# Autodesk Inventor assembly: EX_ONE
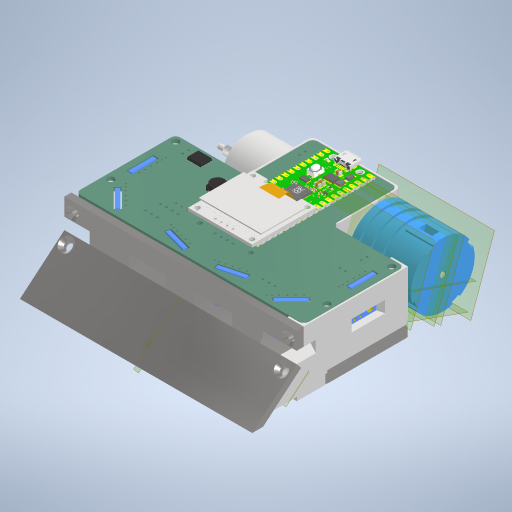
[picture p0: Inventor's stored thumbnail of the model, 512x512]
Saved by Autodesk Inventor 2023.5 (Build 275446000, 446)
## iProperties
Created: 2025-01-11
Part Number: EX_ONE
Document SubType Name: Assembly
Designer: kamil
Author: kamil
## Documents named in this file (17)
- E:\PROJECTS_REPOS\EX_ONE_minisumo\mechanics\inventor_parts\EX_ONE.iam
- E:\PROJECTS_REPOS\EX_ONE_minisumo\mechanics\inventor_parts\faulhaber_motor.ipt
- E:\PROJECTS_REPOS\EX_ONE_minisumo\mechanics\inventor_parts\motors_mount.ipt
- E:\PROJECTS_REPOS\EX_ONE_minisumo\mechanics\inventor_parts\kolo_tetsowe.ipt
- E:\PROJECTS_REPOS\EX_ONE_minisumo\mechanics\inventor_parts\podstawa.ipt
- E:\PROJECTS_REPOS\EX_ONE_minisumo\mechanics\inventor_parts\nóź.ipt
- E:\PROJECTS_REPOS\EX_ONE_minisumo\mechanics\inventor_parts\TOF_VL53L0X (1).ipt
- E:\PROJECTS_REPOS\EX_ONE_minisumo\mechanics\inventor_parts\ściana.ipt
- E:\PROJECTS_REPOS\EX_ONE_minisumo\mechanics\inventor_parts\przod.ipt
- E:\PROJECTS_REPOS\EX_ONE_minisumo\mechanics\inventor_parts\oslona.ipt
- E:\PROJECTS_REPOS\EX_ONE_minisumo\mechanics\inventor_parts\pokrywa.ipt
- E:\PROJECTS_REPOS\EX_ONE_minisumo\mechanics\inventor_parts\belka.ipt
- E:\PROJECTS_REPOS\EX_ONE_minisumo\mechanics\inventor_parts\pcb_czujnik.ipt
- E:\PROJECTS_REPOS\EX_ONE_minisumo\mechanics\inventor_parts\li_po_400mAh.ipt
- E:\PROJECTS_REPOS\EX_ONE_minisumo\mechanics\inventor_parts\main_pcb.ipt
- E:\PROJECTS_REPOS\EX_ONE_minisumo\mechanics\step\main_board_2\main_board_2.iam
- E:\PROJECTS_REPOS\EX_ONE_minisumo\mechanics\inventor_parts\sciana_left.ipt
## Components (24 placed, 16 different names)
1. faulhaber_motor:1 — Zestawiające:31
2. faulhaber_motor:2 — Zestawiające:30
3. motors_mount:1 — Zestawiające:29, Zestawiające:30, Zestawiające:31, Równoległe:53
4. kolo_tetsowe:1
5. nóź:1 — Zestawiające:48
6. kolo_tetsowe:2
7. ściana:1 — Zestawiające:18, Równoległe:21, Zestawiające:19, Równoległe:22, Zestawiające:28, Równoległe:27, Równoległe:28, Równoległe:30, Zestawiające:34, Kątowe:9, Równoległe:35, Zestawiające:35, Zestawiające:43
8. przod:1 — Zestawiające:18, Równoległe:21, Zestawiające:19, Kątowe:6, Zestawiające:22
9. oslona:1 — Równoległe:22, Zestawiające:41
10. pokrywa:1
11. TOF_VL53L0X (1):7 — Kątowe:6, Zestawiające:20, Zestawiające:22, Kątowe:10, Równoległe:47
12. belka:1 — Zestawiające:28, Równoległe:27, Równoległe:28
13. podstawa:1 — Zestawiające:29, Równoległe:30, Zestawiające:40, Zestawiające:47, Równoległe:54
14. pcb_czujnik:1 — Zestawiające:34, Kątowe:9, Równoległe:35, Zestawiające:35
15. li_po_400mAh:1 — Zestawiające:40, Zestawiające:41, Równoległe:53
16. main_pcb:1 — Równoległe:37, Równoległe:39, Równoległe:40, Równoległe:41, Równoległe:42, Zestawiające:36, Zestawiające:37, Zestawiające:39
17. TOF_VL53L0X (1):8 — Równoległe:37
18. TOF_VL53L0X (1):9 — Równoległe:52, Zestawiające:45, Zestawiające:46
19. TOF_VL53L0X (1):10 — Równoległe:40, Zestawiające:39
20. TOF_VL53L0X (1):11 — Równoległe:39, Kątowe:10, Równoległe:47, Zestawiające:36, Równoległe:52
21. TOF_VL53L0X (1):12 — Równoległe:41, Zestawiające:37
22. TOF_VL53L0X (1):13 — Równoległe:42
23. main_board_2:1 [sub-assembly] — Zestawiające:43, Zestawiające:45, Zestawiające:46
24. sciana_left:1 — Zestawiające:47, Zestawiające:48, Równoległe:54
## Relationships (38: Mate 20, Flush 15, Angle 3)
- Zestawiające:18 [Mate]: ściana:1 ↔ przod:1
- Równoległe:21 [Flush]: ściana:1 ↔ przod:1
- Zestawiające:19 [Mate]: ściana:1 ↔ przod:1
- Równoległe:22 [Flush]: ściana:1 ↔ oslona:1
- Kątowe:6 [Angle] (-195 deg): przod:1 ↔ TOF_VL53L0X (1):7
- Zestawiające:20 [Mate] (10 mm): TOF_VL53L0X (1):7
- Zestawiające:22 [Mate] (2 mm): przod:1 ↔ TOF_VL53L0X (1):7
- Zestawiające:28 [Mate]: ściana:1 ↔ belka:1
- Równoległe:27 [Flush]: ściana:1 ↔ belka:1
- Równoległe:28 [Flush]: ściana:1 ↔ belka:1
- Zestawiające:29 [Mate]: motors_mount:1 ↔ podstawa:1
- Równoległe:30 [Flush]: ściana:1 ↔ podstawa:1
- Zestawiające:30 [Mate]: faulhaber_motor:2 ↔ motors_mount:1
- Zestawiające:31 [Mate]: faulhaber_motor:1 ↔ motors_mount:1
- Zestawiające:34 [Mate]: ściana:1 ↔ pcb_czujnik:1
- Kątowe:9 [Angle] (0 deg): ściana:1 ↔ pcb_czujnik:1
- Równoległe:35 [Flush]: ściana:1 ↔ pcb_czujnik:1
- Zestawiające:35 [Mate] (0.5 mm): ściana:1 ↔ pcb_czujnik:1
- Równoległe:37 [Flush]: main_pcb:1 ↔ TOF_VL53L0X (1):8
- Równoległe:39 [Flush]: main_pcb:1 ↔ TOF_VL53L0X (1):11
- Równoległe:40 [Flush]: main_pcb:1 ↔ TOF_VL53L0X (1):10
- Równoległe:41 [Flush]: main_pcb:1 ↔ TOF_VL53L0X (1):12
- Równoległe:42 [Flush]: main_pcb:1 ↔ TOF_VL53L0X (1):13
- Kątowe:10 [Angle] (0 deg): TOF_VL53L0X (1):7 ↔ TOF_VL53L0X (1):11
- Równoległe:47 [Flush]: TOF_VL53L0X (1):7 ↔ TOF_VL53L0X (1):11
- Zestawiające:36 [Mate] (-2 mm): main_pcb:1 ↔ TOF_VL53L0X (1):11
- Zestawiające:37 [Mate] (-2 mm): main_pcb:1 ↔ TOF_VL53L0X (1):12
- Zestawiające:39 [Mate] (-2 mm): main_pcb:1 ↔ TOF_VL53L0X (1):10
- Zestawiające:40 [Mate]: podstawa:1 ↔ li_po_400mAh:1
- Zestawiające:41 [Mate]: oslona:1 ↔ li_po_400mAh:1
- Równoległe:52 [Flush]: TOF_VL53L0X (1):9 ↔ TOF_VL53L0X (1):11
- Równoległe:53 [Flush] (8 mm): motors_mount:1 ↔ li_po_400mAh:1
- Zestawiające:43 [Mate]: ściana:1 ↔ main_board_2:1
- Zestawiające:45 [Mate] (0.5 mm): TOF_VL53L0X (1):9 ↔ main_board_2:1
- Zestawiające:46 [Mate] (0.5 mm): TOF_VL53L0X (1):9 ↔ main_board_2:1
- Zestawiające:47 [Mate]: podstawa:1 ↔ sciana_left:1
- Zestawiające:48 [Mate]: nóź:1 ↔ sciana_left:1
- Równoległe:54 [Flush]: podstawa:1 ↔ sciana_left:1
